# Autodesk Inventor assembly: ElectronGun
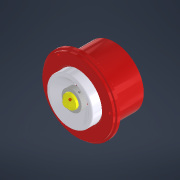
[picture p0: Inventor's stored thumbnail of the model, 180x180]
Saved by Autodesk Inventor 2022 (Build 260153000, 153)
## iProperties
Created: 2022-03-31
Part Number: ElectronGun
Document SubType Name: Assembly
Designer: Vinicius Miguel
Author: Vinicius Miguel
## Documents named in this file (7)
- C:\ViniFiles\SEM-Mechanical\ElectronGun.iam
- C:\ViniFiles\SEM-Mechanical\016.ipt
- C:\ViniFiles\SEM-Mechanical\017.ipt
- C:\ViniFiles\SEM-Mechanical\018.ipt
- C:\ViniFiles\SEM-Mechanical\019.ipt
- C:\ViniFiles\SEM-Mechanical\020.ipt
- C:\ViniFiles\SEM-Mechanical\021.ipt
## Components (6 placed, 6 different names)
1. 016:1 — Mate:1, Mate:2, Mate:3, Mate:5, Rotational:3
2. 017:1 — Rotational:3
3. 018:1 — Mate:4, Mate:5, Flush:1, Rotational:2
4. 019:1 — Rotational:2
5. 020:1 — Rotational:1, Flush:1
6. 021:1 — Mate:6, Rotational:1
## Relationships (10: Mate 6, RevoluteJoint 3, Flush 1)
- Mate:1: 016:1
- Mate:2: 016:1
- Mate:3: 016:1
- Mate:4: 018:1
- Mate:5: 016:1 ↔ 018:1
- Mate:6: 021:1
- Rotational:1 [RevoluteJoint]: 020:1 ↔ 021:1
- Flush:1: 018:1 ↔ 020:1
- Rotational:2 [RevoluteJoint]: 018:1 ↔ 019:1
- Rotational:3 [RevoluteJoint]: 016:1 ↔ 017:1
